# Autodesk Inventor assembly: splitter_all
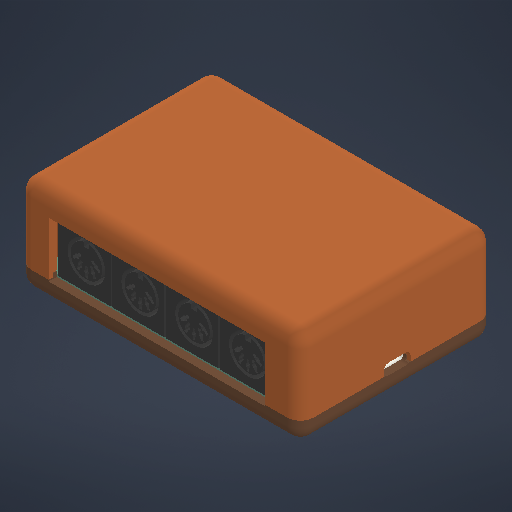
[picture p0: Inventor's stored thumbnail of the model, 512x512]
Saved by Autodesk Inventor 2025.2 (Build 292293000, 293)
## iProperties
Created: 2025-10-04
Part Number: splitter_all
Document SubType Name: Assembly
Designer: micyg
Author: micyg
## Documents named in this file (4)
- D:\Projects\AnotherMidiSplitterV2\Mechanical\splitter_all.iam
- D:\Projects\AnotherMidiSplitterV2\Mechanical\Boards\AnotherMidiSplitterV2\AnotherMidiSplitterV2.iam
- D:\Projects\AnotherMidiSplitterV2\Mechanical\case1.ipt
- D:\Projects\AnotherMidiSplitterV2\Mechanical\case2.ipt
## Components (3 placed, 3 different names)
1. AnotherMidiSplitterV2:1 [sub-assembly] — Mate:3, Mate:4, Mate:5
2. case1:1 — Mate:3, Mate:4, Mate:5, Mate:6, Flush:1, Flush:2
3. case2:1 — Mate:6, Flush:1, Flush:2
## Relationships (6: Mate 4, Flush 2)
- Mate:3: AnotherMidiSplitterV2:1 ↔ case1:1
- Mate:4: AnotherMidiSplitterV2:1 ↔ case1:1
- Mate:5: AnotherMidiSplitterV2:1 ↔ case1:1
- Mate:6: case1:1 ↔ case2:1
- Flush:1: case1:1 ↔ case2:1
- Flush:2: case1:1 ↔ case2:1
